# Autodesk Inventor assembly: center2
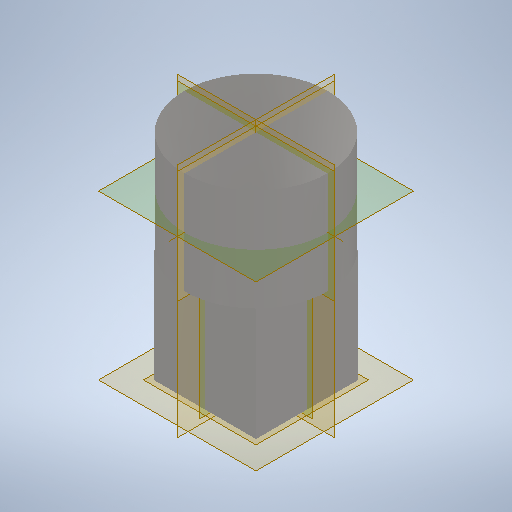
[picture p0: Inventor's stored thumbnail of the model, 512x512]
Saved by Autodesk Inventor 2025.2 (Build 292293000, 293)
## iProperties
Created: 2025-06-19
Part Number: center2
Document SubType Name: Assembly
Designer: MSIGAMING
Author: MSIGAMING
## Documents named in this file (3)
- D:\One Drive Manuel\OneDrive\21 Master APE\II Semester\Robotik\3d_robotik\center2.iam
- D:\One Drive Manuel\OneDrive\21 Master APE\II Semester\Robotik\3d_robotik\D1_lenght.ipt
- D:\One Drive Manuel\OneDrive\21 Master APE\II Semester\Robotik\3d_robotik\Gelenk 2.ipt
## Components (2 placed, 2 different names)
1. D1_lenght:1 — Mate:1, Mate:2, Flush:1, Mate:3
2. Gelenk 2:1 — Mate:3, Mate:4, Flush:2
## Relationships (6: Mate 4, Flush 2)
- Mate:1: D1_lenght:1
- Mate:2: D1_lenght:1
- Flush:1: D1_lenght:1
- Mate:3: D1_lenght:1 ↔ Gelenk 2:1
- Mate:4: Gelenk 2:1
- Flush:2: Gelenk 2:1
